# Autodesk Inventor assembly: Montagem estação para fixação sem tripé v1
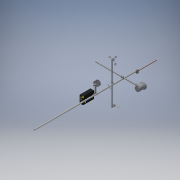
[picture p0: Inventor's stored thumbnail of the model, 180x180]
Saved by Autodesk Inventor 2019.4 (Build 234330000, 330)
## iProperties
Created: 2021-02-17
Part Number: Montagem estação para fixação sem tripé v1
Material: Genérico
Document SubType Name: Assembly
Designer: Lattes
Author: Lattes
## Documents named in this file (18)
- D:\Lattes\Documents\GitHub-HD\estacao-meteorologica-it\Estuturas\Montagem estação para fixação sem tripé v1.iam
- D:\Lattes\Documents\GitHub-HD\estacao-meteorologica-it\Estuturas\Tubo 32x2500mm.ipt
- D:\Lattes\Documents\GitHub-HD\estacao-meteorologica-it\Estuturas\caixa\caixa de instrumentação e controle.iam
- D:\Lattes\Documents\GitHub-HD\estacao-meteorologica-it\Estuturas\anemometro.ipt
- D:\Lattes\Documents\GitHub-HD\estacao-meteorologica-it\Estuturas\porca m3.ipt
- D:\Lattes\Documents\GitHub-HD\estacao-meteorologica-it\Estuturas\wind_vane.ipt
- D:\Lattes\Documents\GitHub-HD\estacao-meteorologica-it\Estuturas\Alojamento do Sensor de Temperatura e Umidade\alojamento sensor temperatura.iam
- D:\Lattes\Documents\GitHub-HD\estacao-meteorologica-it\Estuturas\pluviometro.ipt
- D:\Lattes\Documents\GitHub-HD\estacao-meteorologica-it\Estuturas\0070.2 - Abraçadeira suporte.ipt
- D:\Lattes\Documents\GitHub-HD\estacao-meteorologica-it\Estuturas\0070.1 - Abraçadeira U Vergalhão bitola 1 polegada 80mm rosca 1 quarto.ipt
- D:\Lattes\Documents\GitHub-HD\estacao-meteorologica-it\Estuturas\Haste para-raio.ipt
- D:\Lattes\Documents\GitHub-HD\estacao-meteorologica-it\Estuturas\Porca sextavada 1 quarto.ipt
- D:\Lattes\Documents\GitHub-HD\estacao-meteorologica-it\Estuturas\Ruela lisa para 1 quarto.ipt
- D:\Lattes\Documents\GitHub-HD\estacao-meteorologica-it\Estuturas\Haste anemometro e wind vane.ipt
- D:\Lattes\Documents\GitHub-HD\estacao-meteorologica-it\Estuturas\Haste pluviômetro e sensores solares.ipt
- D:\Lattes\Documents\GitHub-HD\estacao-meteorologica-it\Estuturas\Parafuso sextavado 1 quarto 30mm.ipt
- D:\Lattes\Documents\GitHub-HD\estacao-meteorologica-it\Estuturas\barra roscada 100 mm rosca 1 quarto.ipt
- D:\Lattes\Documents\GitHub-HD\estacao-meteorologica-it\Estuturas\Parafuso m5 16mm.ipt
## Components (66 placed, 17 different names)
1. Tubo 32x2500mm:1 — Inserir:40, Coincidência:1, Tangente:2, Inserir:95, Inserir:96, Inserir:105
2. porca m3:1 — Inserir:78
3. anemometro:1 — Inserir:76
4. wind_vane:1 — Inserir:79
5. porca m3:2 — Inserir:77
6. caixa de instrumentação e controle:2 [sub-assembly] — Inserir:40, Inserir:115, Inserir:116, Inserir:117, Inserir:118
7. pluviometro:1 — Inserir:89, Coincidência:4, Inserir:90
8. 0070.2 - Abraçadeira suporte:1 — Inserir:58, Coincidência:2, Alinhamento:1, Alinhamento:2, Tangente:1, Alinhamento:3, Tangente:3, Tangente:4, Inserir:62, Inserir:63
9. 0070.1 - Abraçadeira U Vergalhão bitola 1 polegada 80mm rosca 1 quarto:1 — Coincidência:1, Inserir:58
10. 0070.2 - Abraçadeira suporte:2 — Coincidência:2, Alinhamento:1, Alinhamento:2, Alinhamento:4, Inserir:59, Inserir:64, Inserir:65
11. Haste para-raio:1 — Tangente:1, Alinhamento:3, Tangente:2, Alinhamento:4, Tangente:3, Tangente:4
12. 0070.1 - Abraçadeira U Vergalhão bitola 1 polegada 80mm rosca 1 quarto:2 — Inserir:59
13. 0070.1 - Abraçadeira U Vergalhão bitola 1 polegada 80mm rosca 1 quarto:3 — Inserir:60, Inserir:84
14. 0070.2 - Abraçadeira suporte:3 — Inserir:60
15. Porca sextavada 1 quarto:1 — Inserir:71
16. Porca sextavada 1 quarto:2 — Inserir:73
17. Porca sextavada 1 quarto:3 — Inserir:72
18. Porca sextavada 1 quarto:4 — Inserir:70
19. Ruela lisa para 1 quarto:1 — Inserir:64, Inserir:73
20. Ruela lisa para 1 quarto:2 — Inserir:65, Inserir:72
21. Ruela lisa para 1 quarto:3 — Inserir:62, Inserir:70
22. Ruela lisa para 1 quarto:4 — Inserir:63, Inserir:71
23. 0070.1 - Abraçadeira U Vergalhão bitola 1 polegada 80mm rosca 1 quarto:4 — Inserir:74
24. Haste anemometro e wind vane:1 — Inserir:74, Inserir:75, Coincidência:3, Inserir:76, Inserir:77, Inserir:78, Inserir:79, Inserir:80, Inserir:81
25. 0070.2 - Abraçadeira suporte:4 — Inserir:75, Coincidência:3
26. Ruela lisa para 1 quarto:8 — Inserir:81, Inserir:82
27. Ruela lisa para 1 quarto:9 — Inserir:80, Inserir:83
28. Porca sextavada 1 quarto:7 — Inserir:83
29. Porca sextavada 1 quarto:8 — Inserir:82
30. Haste pluviômetro e sensores solares:2 — Inserir:84, Inserir:85, Inserir:86, Inserir:89, Inserir:91, Inserir:92
31. Ruela lisa para 1 quarto:10 — Inserir:85, Inserir:87
32. Ruela lisa para 1 quarto:11 — Inserir:86, Inserir:88
33. Porca sextavada 1 quarto:9 — Inserir:87
34. Porca sextavada 1 quarto:10 — Inserir:88
35. Parafuso sextavado 1 quarto 30mm:1 — Inserir:90
36. Parafuso sextavado 1 quarto 30mm:2 — Coincidência:4
37. Ruela lisa para 1 quarto:12 — Inserir:92, Inserir:93
38. Ruela lisa para 1 quarto:13 — Inserir:91, Inserir:94
39. Porca sextavada 1 quarto:11 — Inserir:94
40. Porca sextavada 1 quarto:12 — Inserir:93
41. barra roscada 100 mm rosca 1 quarto:2 — Inserir:95, Inserir:101, Inserir:102, Inserir:103, Inserir:104, Inserir:111, Inserir:112
42. barra roscada 100 mm rosca 1 quarto:3 — Inserir:96, Inserir:97, Inserir:98, Inserir:99, Inserir:100, Inserir:113, Inserir:114
43. Porca sextavada 1 quarto:13 — Inserir:101
44. Porca sextavada 1 quarto:14 — Inserir:103
45. Porca sextavada 1 quarto:15 — Inserir:104
46. Porca sextavada 1 quarto:16 — Inserir:102
47. Porca sextavada 1 quarto:17 — Inserir:98
48. Porca sextavada 1 quarto:18 — Inserir:99
49. Porca sextavada 1 quarto:19 — Inserir:100
50. Porca sextavada 1 quarto:20 — Inserir:97
51. alojamento sensor temperatura:1 [sub-assembly] — Inserir:105, Inserir:106, Inserir:107, Inserir:108
52. 0070.1 - Abraçadeira U Vergalhão bitola 1 polegada 80mm rosca 1 quarto:5 — Inserir:106
53. Ruela lisa para 1 quarto:14 — Inserir:108, Inserir:110
54. Ruela lisa para 1 quarto:15 — Inserir:107, Inserir:109
55. Porca sextavada 1 quarto:21 — Inserir:109
56. Porca sextavada 1 quarto:22 — Inserir:110
57. Ruela lisa para 1 quarto:16 — Inserir:114
58. Ruela lisa para 1 quarto:17 — Inserir:112
59. Ruela lisa para 1 quarto:18 — Inserir:111
60. Ruela lisa para 1 quarto:19 — Inserir:113
61. Parafuso m5 16mm:1 — Inserir:115
62. 0070.1 - Abraçadeira U Vergalhão bitola 1 polegada 80mm rosca 1 quarto:6 — Inserir:116
63. Ruela lisa para 1 quarto:20 — Inserir:117, Inserir:119
64. Ruela lisa para 1 quarto:21 — Inserir:118, Inserir:120
65. Porca sextavada 1 quarto:23 — Inserir:119
66. Porca sextavada 1 quarto:24 — Inserir:120
## Relationships (71: Insert 59, Mate 4, Flush 4, Tangent 4)
- Inserir:40: Tubo 32x2500mm:1 ↔ caixa de instrumentação e controle:2
- Coincidência:1 [Mate] (-1.35 mm): Tubo 32x2500mm:1 ↔ 0070.1 - Abraçadeira U Vergalhão bitola 1 polegada 80mm rosca 1 quarto:1
- Inserir:58 (-28.4 mm): 0070.2 - Abraçadeira suporte:1 ↔ 0070.1 - Abraçadeira U Vergalhão bitola 1 polegada 80mm rosca 1 quarto:1
- Coincidência:2 [Mate] (10 mm): 0070.2 - Abraçadeira suporte:1 ↔ 0070.2 - Abraçadeira suporte:2
- Alinhamento:1 [Flush]: 0070.2 - Abraçadeira suporte:1 ↔ 0070.2 - Abraçadeira suporte:2
- Alinhamento:2 [Flush]: 0070.2 - Abraçadeira suporte:1 ↔ 0070.2 - Abraçadeira suporte:2
- Tangente:1 (5 mm): 0070.2 - Abraçadeira suporte:1 ↔ Haste para-raio:1
- Alinhamento:3 [Flush]: 0070.2 - Abraçadeira suporte:1 ↔ Haste para-raio:1
- Tangente:2: Tubo 32x2500mm:1 ↔ Haste para-raio:1
- Alinhamento:4 [Flush] (-10 mm): 0070.2 - Abraçadeira suporte:2 ↔ Haste para-raio:1
- Tangente:3 (4.5 mm): 0070.2 - Abraçadeira suporte:1 ↔ Haste para-raio:1
- Tangente:4: 0070.2 - Abraçadeira suporte:1 ↔ Haste para-raio:1
- Inserir:59 (-28.4 mm): 0070.2 - Abraçadeira suporte:2 ↔ 0070.1 - Abraçadeira U Vergalhão bitola 1 polegada 80mm rosca 1 quarto:2
- Inserir:60 (-37.6 mm): 0070.1 - Abraçadeira U Vergalhão bitola 1 polegada 80mm rosca 1 quarto:3 ↔ 0070.2 - Abraçadeira suporte:3
- Inserir:62: 0070.2 - Abraçadeira suporte:1 ↔ Ruela lisa para 1 quarto:3
- Inserir:63: 0070.2 - Abraçadeira suporte:1 ↔ Ruela lisa para 1 quarto:4
- Inserir:64: 0070.2 - Abraçadeira suporte:2 ↔ Ruela lisa para 1 quarto:1
- Inserir:65: 0070.2 - Abraçadeira suporte:2 ↔ Ruela lisa para 1 quarto:2
- Inserir:70: Porca sextavada 1 quarto:4 ↔ Ruela lisa para 1 quarto:3
- Inserir:71: Porca sextavada 1 quarto:1 ↔ Ruela lisa para 1 quarto:4
- Inserir:72: Porca sextavada 1 quarto:3 ↔ Ruela lisa para 1 quarto:2
- Inserir:73: Porca sextavada 1 quarto:2 ↔ Ruela lisa para 1 quarto:1
- Inserir:74 (-35 mm): 0070.1 - Abraçadeira U Vergalhão bitola 1 polegada 80mm rosca 1 quarto:4 ↔ Haste anemometro e wind vane:1
- Inserir:75 (5 mm): Haste anemometro e wind vane:1 ↔ 0070.2 - Abraçadeira suporte:4
- Coincidência:3 [Mate]: Haste anemometro e wind vane:1 ↔ 0070.2 - Abraçadeira suporte:4
- Inserir:76: anemometro:1 ↔ Haste anemometro e wind vane:1
- Inserir:77: porca m3:2 ↔ Haste anemometro e wind vane:1
- Inserir:78: porca m3:1 ↔ Haste anemometro e wind vane:1
- Inserir:79: wind_vane:1 ↔ Haste anemometro e wind vane:1
- Inserir:80: Haste anemometro e wind vane:1 ↔ Ruela lisa para 1 quarto:9
- Inserir:81: Haste anemometro e wind vane:1 ↔ Ruela lisa para 1 quarto:8
- Inserir:82: Ruela lisa para 1 quarto:8 ↔ Porca sextavada 1 quarto:8
- Inserir:83: Ruela lisa para 1 quarto:9 ↔ Porca sextavada 1 quarto:7
- Inserir:84 (-35.6 mm): 0070.1 - Abraçadeira U Vergalhão bitola 1 polegada 80mm rosca 1 quarto:3 ↔ Haste pluviômetro e sensores solares:2
- Inserir:85: Haste pluviômetro e sensores solares:2 ↔ Ruela lisa para 1 quarto:10
- Inserir:86: Haste pluviômetro e sensores solares:2 ↔ Ruela lisa para 1 quarto:11
- Inserir:87: Ruela lisa para 1 quarto:10 ↔ Porca sextavada 1 quarto:9
- Inserir:88: Ruela lisa para 1 quarto:11 ↔ Porca sextavada 1 quarto:10
- Inserir:89: pluviometro:1 ↔ Haste pluviômetro e sensores solares:2
- Coincidência:4 [Mate]: pluviometro:1 ↔ Parafuso sextavado 1 quarto 30mm:2
- Inserir:90: pluviometro:1 ↔ Parafuso sextavado 1 quarto 30mm:1
- Inserir:91: Haste pluviômetro e sensores solares:2 ↔ Ruela lisa para 1 quarto:13
- Inserir:92: Haste pluviômetro e sensores solares:2 ↔ Ruela lisa para 1 quarto:12
- Inserir:93: Ruela lisa para 1 quarto:12 ↔ Porca sextavada 1 quarto:12
- Inserir:94: Ruela lisa para 1 quarto:13 ↔ Porca sextavada 1 quarto:11
- Inserir:95 (-66 mm): Tubo 32x2500mm:1 ↔ barra roscada 100 mm rosca 1 quarto:2
- Inserir:96 (-66 mm): Tubo 32x2500mm:1 ↔ barra roscada 100 mm rosca 1 quarto:3
- Inserir:97 (-34 mm): barra roscada 100 mm rosca 1 quarto:3 ↔ Porca sextavada 1 quarto:20
- Inserir:98 (-34 mm): barra roscada 100 mm rosca 1 quarto:3 ↔ Porca sextavada 1 quarto:17
- Inserir:99 (-10 mm): barra roscada 100 mm rosca 1 quarto:3 ↔ Porca sextavada 1 quarto:18
- Inserir:100 (-10 mm): barra roscada 100 mm rosca 1 quarto:3 ↔ Porca sextavada 1 quarto:19
- Inserir:101 (-34.5 mm): barra roscada 100 mm rosca 1 quarto:2 ↔ Porca sextavada 1 quarto:13
- Inserir:102 (-33.5 mm): barra roscada 100 mm rosca 1 quarto:2 ↔ Porca sextavada 1 quarto:16
- Inserir:103 (-10 mm): barra roscada 100 mm rosca 1 quarto:2 ↔ Porca sextavada 1 quarto:14
- Inserir:104 (-10 mm): barra roscada 100 mm rosca 1 quarto:2 ↔ Porca sextavada 1 quarto:15
- Inserir:105: Tubo 32x2500mm:1 ↔ alojamento sensor temperatura:1
- Inserir:106 (-44 mm): alojamento sensor temperatura:1 ↔ 0070.1 - Abraçadeira U Vergalhão bitola 1 polegada 80mm rosca 1 quarto:5
- Inserir:107: alojamento sensor temperatura:1 ↔ Ruela lisa para 1 quarto:15
- Inserir:108: alojamento sensor temperatura:1 ↔ Ruela lisa para 1 quarto:14
- Inserir:109: Ruela lisa para 1 quarto:15 ↔ Porca sextavada 1 quarto:21
- Inserir:110: Ruela lisa para 1 quarto:14 ↔ Porca sextavada 1 quarto:22
- Inserir:111 (-20 mm): barra roscada 100 mm rosca 1 quarto:2 ↔ Ruela lisa para 1 quarto:18
- Inserir:112 (-20 mm): barra roscada 100 mm rosca 1 quarto:2 ↔ Ruela lisa para 1 quarto:17
- Inserir:113 (-20 mm): barra roscada 100 mm rosca 1 quarto:3 ↔ Ruela lisa para 1 quarto:19
- Inserir:114 (-20 mm): barra roscada 100 mm rosca 1 quarto:3 ↔ Ruela lisa para 1 quarto:16
- Inserir:115: caixa de instrumentação e controle:2 ↔ Parafuso m5 16mm:1
- Inserir:116 (-43 mm): caixa de instrumentação e controle:2 ↔ 0070.1 - Abraçadeira U Vergalhão bitola 1 polegada 80mm rosca 1 quarto:6
- Inserir:117: caixa de instrumentação e controle:2 ↔ Ruela lisa para 1 quarto:20
- Inserir:118: caixa de instrumentação e controle:2 ↔ Ruela lisa para 1 quarto:21
- Inserir:119: Ruela lisa para 1 quarto:20 ↔ Porca sextavada 1 quarto:23
- Inserir:120: Ruela lisa para 1 quarto:21 ↔ Porca sextavada 1 quarto:24
